# Autodesk Inventor assembly: Assembly3
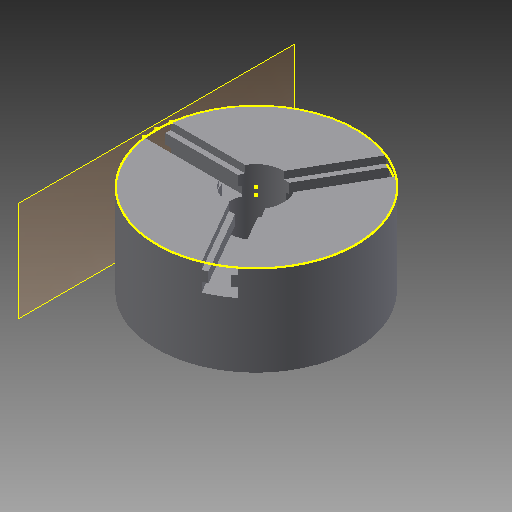
[picture p0: Inventor's stored thumbnail of the model, 512x512]
Saved by Autodesk Inventor 2018 (Build 220112000, 112)
## iProperties
Created: 2017-06-27
Part Number: Assembly3
Document SubType Name: Assembly
Designer: M228854
Author: M228854
## Documents named in this file (3)
- C:\Users\P301319\Documents\GitHub\CNC-Lathe-CAD\Chucks\3 jaw\Assembly3.iam
- C:\Users\P301319\Documents\GitHub\CNC-Lathe-CAD\Chucks\3 jaw\3 jaww.ipt
- C:\Users\P301319\Documents\GitHub\CNC-Lathe-CAD\Chucks\3 jaw\rod.ipt
## Components (4 placed, 2 different names)
1. 3 jaww:1 — Mate:4, Mate:6, Mate:7
2. rod:6 — Mate:4
3. rod:8 — Mate:6
4. rod:9 — Mate:7
## Relationships (3: Mate 3)
- Mate:4: 3 jaww:1 ↔ rod:6
- Mate:6: 3 jaww:1 ↔ rod:8
- Mate:7: 3 jaww:1 ↔ rod:9
